# Autodesk Inventor assembly: mainASM
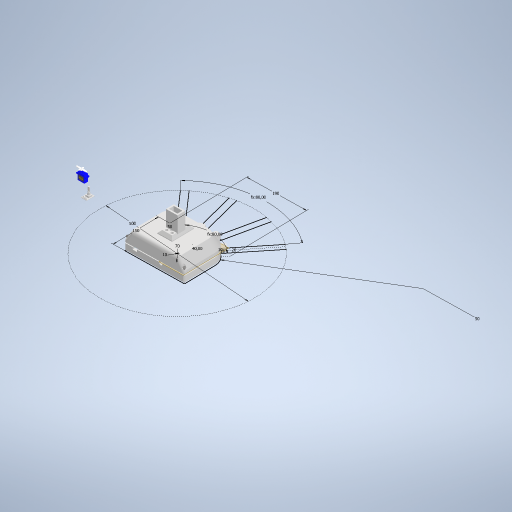
[picture p0: Inventor's stored thumbnail of the model, 512x512]
Saved by Autodesk Inventor 2024.2 (Build 282272000, 272)
## iProperties
Created: 2024-03-11
Part Number: mainASM
Document SubType Name: Assembly
Designer: Daniel
Author: Daniel
## Documents named in this file (11)
- C:\Users\Daniel\Desktop\pmik_2024l_jd\mechanical\mainASM.iam
- C:\Users\Daniel\Desktop\pmik_2024l_jd\mechanical\STEPS\NUCLEO-F091RC.iam
- C:\Users\Daniel\Desktop\pmik_2024l_jd\mechanical\STEPS\SG90 - Micro Servo 9g - Tower Pro.iam
- C:\Users\Daniel\Desktop\pmik_2024l_jd\mechanical\STEPS\KY-040 Rotary Encoder.iam
- C:\Users\Daniel\Desktop\pmik_2024l_jd\mechanical\bottom.ipt
- C:\Users\Daniel\Desktop\pmik_2024l_jd\mechanical\Pump.ipt
- C:\Users\Daniel\Desktop\pmik_2024l_jd\mechanical\STEPS\LM2596 DC to DC Buck Converter 3 A.iam
- C:\Users\Daniel\Desktop\pmik_2024l_jd\mechanical\Top.ipt
- C:\Users\Daniel\Desktop\pmik_2024l_jd\mechanical\Tower.ipt
- C:\Users\Daniel\Documents\Inventor\Content Center Files\R2024\pl-PL\M\M 4x30.ipt
- C:\Users\Daniel\Documents\Inventor\Content Center Files\R2024\pl-PL\M\M 3x10.ipt
## Components (19 placed, 10 different names)
1. NUCLEO-F091RC:1 [sub-assembly] — Zestawiające:3, Zestawiające:4, Zestawiające:5, Obrotowe:5, Obrotowe:6
2. SG90 - Micro Servo 9g - Tower Pro:1 [sub-assembly]
3. KY-040 Rotary Encoder:1 [sub-assembly]
4. bottom:1 — Równoległe:1, Kątowe:1, Zestawiające:3, Zestawiające:4, Zestawiające:5, Zestawiające:6, Zestawiające:7, Zestawiające:8, Zestawiające:9, Równoległe:2, Równoległe:3, Równoległe:4, Równoległe:5
5. Pump:1 — Kątowe:1, Zestawiające:6, Zestawiające:7, Zestawiające:8
6. LM2596 DC to DC Buck Converter 3 A:1 [sub-assembly] — Zestawiające:9, Równoległe:2, Równoległe:3, Obrotowe:3, Obrotowe:4
7. Top:1 — Równoległe:4, Równoległe:5, Obrotowe:1, Obrotowe:2, Sztywne:1, Równoległe:6, Równoległe:7
8. M 4x30:12 — Obrotowe:2
9. M 4x30:13 — Sztywne:1
10. M 4x30:14 — Obrotowe:1
11. M 3x10:5 — Obrotowe:4
12. M 3x10:6 — Obrotowe:3
13. M 3x10:7 — Obrotowe:5
14. M 3x10:8 — Obrotowe:6
15. Tower:1 — Równoległe:6, Równoległe:7, Obrotowe:7, Obrotowe:8, Obrotowe:9, Obrotowe:10
16. M 4x30:8 — Obrotowe:7
17. M 4x30:9 — Obrotowe:8
18. M 4x30:10 — Obrotowe:9
19. M 4x30:11 — Obrotowe:10
## Relationships (26: RevoluteJoint 10, Flush 7, Mate 7, Angle 1, WeldJoint 1)
- Równoległe:1 [Flush]: bottom:1
- Kątowe:1 [Angle] (180 deg): bottom:1 ↔ Pump:1
- Zestawiające:3 [Mate] (3 mm): NUCLEO-F091RC:1 ↔ bottom:1
- Zestawiające:4 [Mate] (2 mm): NUCLEO-F091RC:1 ↔ bottom:1
- Zestawiające:5 [Mate] (5 mm): NUCLEO-F091RC:1 ↔ bottom:1
- Zestawiające:6 [Mate] (25 mm): bottom:1 ↔ Pump:1
- Zestawiające:7 [Mate] (5 mm): bottom:1 ↔ Pump:1
- Zestawiające:8 [Mate] (3 mm): bottom:1 ↔ Pump:1
- Zestawiające:9 [Mate] (5 mm): bottom:1 ↔ LM2596 DC to DC Buck Converter 3 A:1
- Równoległe:2 [Flush] (5 mm): bottom:1 ↔ LM2596 DC to DC Buck Converter 3 A:1
- Równoległe:3 [Flush] (4 mm): bottom:1 ↔ LM2596 DC to DC Buck Converter 3 A:1
- Równoległe:4 [Flush]: bottom:1 ↔ Top:1
- Równoległe:5 [Flush]: bottom:1 ↔ Top:1
- Obrotowe:1 [RevoluteJoint]: Top:1 ↔ M 4x30:14
- Obrotowe:2 [RevoluteJoint]: Top:1 ↔ M 4x30:12
- Sztywne:1 [WeldJoint]: Top:1 ↔ M 4x30:13
- Obrotowe:3 [RevoluteJoint]: LM2596 DC to DC Buck Converter 3 A:1 ↔ M 3x10:6
- Obrotowe:4 [RevoluteJoint]: LM2596 DC to DC Buck Converter 3 A:1 ↔ M 3x10:5
- Obrotowe:5 [RevoluteJoint]: NUCLEO-F091RC:1 ↔ M 3x10:7
- Obrotowe:6 [RevoluteJoint]: NUCLEO-F091RC:1 ↔ M 3x10:8
- Równoległe:6 [Flush]: Top:1 ↔ Tower:1
- Równoległe:7 [Flush]: Top:1 ↔ Tower:1
- Obrotowe:7 [RevoluteJoint]: Tower:1 ↔ M 4x30:8
- Obrotowe:8 [RevoluteJoint]: Tower:1 ↔ M 4x30:9
- Obrotowe:9 [RevoluteJoint]: Tower:1 ↔ M 4x30:10
- Obrotowe:10 [RevoluteJoint]: Tower:1 ↔ M 4x30:11
